# Autodesk Inventor assembly: Cube (Sample)
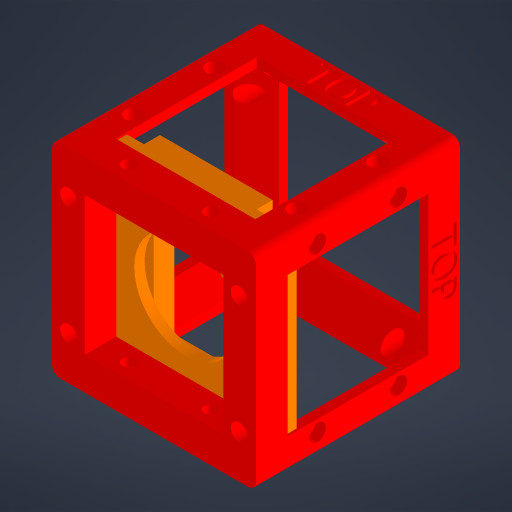
[picture p0: Inventor's stored thumbnail of the model, 512x512]
Saved by Autodesk Inventor 2023.4 (Build 274418000, 418)
## iProperties
Created: 2021-11-17
Part Number: Cube (Sample)
Document SubType Name: Assembly
Designer: xSibe
Author: xSibe
## Documents named in this file (4)
- C:\.Laptop\.Work\Projects\Project Protocube\1 Autodesk\1 Cubes\Sample\Cube (Sample).iam
- C:\.Laptop\.Work\Projects\Project Protocube\1 Autodesk\1 Cubes\Sample\Sample Clamp.ipt
- C:\.Laptop\.Work\Projects\Project Protocube\1 Autodesk\1 Cubes\Sample\Sample Holder.ipt
- C:\.Laptop\.Work\Projects\Project Protocube\1 Autodesk\1 Cubes\Cubes\Cube 1x1 V5.iam
## Components (3 placed, 3 different names)
1. Sample Holder:1 — Flush:3, Flush:4, Flush:5
2. Sample Clamp:1 — Flush:3, Flush:4, Flush:5
3. Cube 1x1 V5:1 [sub-assembly]
## Relationships (3: Flush 3)
- Flush:3: Sample Holder:1 ↔ Sample Clamp:1
- Flush:4: Sample Holder:1 ↔ Sample Clamp:1
- Flush:5: Sample Holder:1 ↔ Sample Clamp:1
